# Autodesk Inventor assembly: Roof
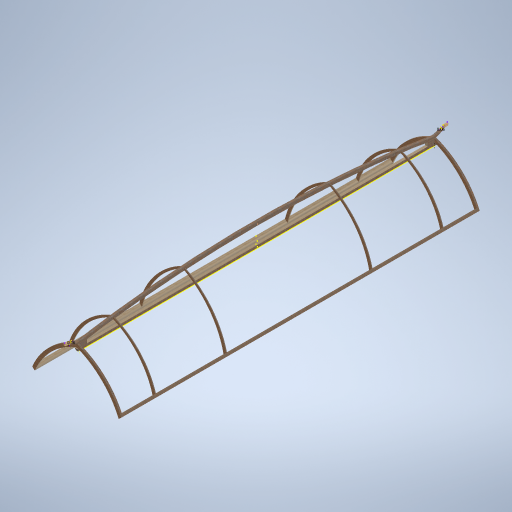
[picture p0: Inventor's stored thumbnail of the model, 512x512]
Saved by Autodesk Inventor 2024.2 (Build 282272000, 272)
## iProperties
Created: 2024-05-18
Part Number: Roof
Document SubType Name: Assembly
Designer: LOSTER_1
Author: LOSTER_1
## Documents named in this file (8)
- C:\Users\LOSTER_1\OneDrive\桌面\school\senior\Inventor_Project\ROOF\Roof.iam
- C:\Users\LOSTER_1\OneDrive\桌面\school\senior\Inventor_Project\ROOF\roof_beam.ipt
- C:\Users\LOSTER_1\OneDrive\桌面\school\senior\Inventor_Project\ROOF\gripping_beast.ipt
- C:\Users\LOSTER_1\OneDrive\桌面\school\senior\Inventor_Project\ROOF\main_crossbeam.ipt
- C:\Users\LOSTER_1\OneDrive\桌面\school\senior\Inventor_Project\ROOF\outer_curve_beam.ipt
- C:\Users\LOSTER_1\OneDrive\桌面\school\senior\Inventor_Project\ROOF\roof_straight_beam.ipt
- C:\Users\LOSTER_1\OneDrive\桌面\school\senior\Inventor_Project\ROOF\curve_beam_01.ipt
- C:\Users\LOSTER_1\OneDrive\桌面\school\senior\Inventor_Project\ROOF\curve_beam_02.ipt
## Components (18 placed, 7 different names)
1. roof_beam:1 — Mate:1, Mate:2, Mate:3, Mate:4, Mate:5, Mate:6, Mate:7, Mate:8, Mate:31, Mate:32, Mate:33, Mate:34, Mate:35, Mate:36, Mate:37, Mate:38, Mate:39, Mate:40, Mate:41, Mate:42, Mate:43, Mate:44, Mate:45, Mate:46, Mate:47, Mate:48, Mate:49, Mate:50
2. gripping_beast:1 — Mate:1, Mate:2, Mate:3, Mate:4
3. gripping_beast:2 — Mate:5
4. main_crossbeam:1 — Mate:6, Mate:7, Mate:8, Mate:11, Mate:14, Mate:19, Mate:20, Mate:21, Mate:22
5. outer_curve_beam:1 — Mate:9, Mate:10, Mate:11, Mate:12, Mate:13, Mate:26, Mate:28
6. outer_curve_beam:2 — Mate:9, Mate:10, Mate:12, Mate:13, Mate:14, Mate:29, Mate:30
7. outer_curve_beam:3 — Mate:23, Mate:24, Mate:25, Mate:27
8. outer_curve_beam:4 — Mate:19, Mate:20, Mate:21, Mate:22, Mate:23, Mate:24, Mate:25
9. roof_straight_beam:1 — Mate:26, Mate:27, Mate:28
10. roof_straight_beam:2 — Mate:29, Mate:30
11. curve_beam_01:1 — Mate:31, Mate:32, Mate:33
12. curve_beam_01:2 — Mate:34, Mate:35
13. curve_beam_01:3 — Mate:36, Mate:37
14. curve_beam_01:4 — Mate:38, Mate:39
15. curve_beam_02:1 — Mate:43, Mate:44
16. curve_beam_02:2 — Mate:40, Mate:41, Mate:42
17. curve_beam_02:3 — Mate:45, Mate:46, Mate:47
18. curve_beam_02:4 — Mate:48, Mate:49, Mate:50
## Relationships (50: Mate 50)
- Mate:1: roof_beam:1 ↔ gripping_beast:1
- Mate:2: roof_beam:1 ↔ gripping_beast:1
- Mate:3: roof_beam:1 ↔ gripping_beast:1
- Mate:4: roof_beam:1 ↔ gripping_beast:1
- Mate:5: roof_beam:1 ↔ gripping_beast:2
- Mate:6: roof_beam:1 ↔ main_crossbeam:1
- Mate:7: roof_beam:1 ↔ main_crossbeam:1
- Mate:8: roof_beam:1 ↔ main_crossbeam:1
- Mate:9: outer_curve_beam:1 ↔ outer_curve_beam:2
- Mate:10: outer_curve_beam:1 ↔ outer_curve_beam:2
- Mate:11: main_crossbeam:1 ↔ outer_curve_beam:1
- Mate:12: outer_curve_beam:1 ↔ outer_curve_beam:2
- Mate:13: outer_curve_beam:1 ↔ outer_curve_beam:2
- Mate:14: main_crossbeam:1 ↔ outer_curve_beam:2
- [Mate]: outer_curve_beam:3 ↔ outer_curve_beam:4
- [Mate]: outer_curve_beam:3 ↔ outer_curve_beam:4
- [Mate]: outer_curve_beam:3 ↔ outer_curve_beam:4
- [Mate]: outer_curve_beam:3 ↔ outer_curve_beam:4
- Mate:19: main_crossbeam:1 ↔ outer_curve_beam:4
- Mate:20: main_crossbeam:1 ↔ outer_curve_beam:4
- Mate:21: main_crossbeam:1 ↔ outer_curve_beam:4
- Mate:22: main_crossbeam:1 ↔ outer_curve_beam:4
- Mate:23: outer_curve_beam:3 ↔ outer_curve_beam:4
- Mate:24: outer_curve_beam:3 ↔ outer_curve_beam:4
- Mate:25: outer_curve_beam:3 ↔ outer_curve_beam:4
- Mate:26: outer_curve_beam:1 ↔ roof_straight_beam:1
- Mate:27: outer_curve_beam:3 ↔ roof_straight_beam:1
- Mate:28: outer_curve_beam:1 ↔ roof_straight_beam:1
- Mate:29: outer_curve_beam:2 ↔ roof_straight_beam:2
- Mate:30: outer_curve_beam:2 ↔ roof_straight_beam:2
- Mate:31: roof_beam:1 ↔ curve_beam_01:1
- Mate:32: roof_beam:1 ↔ curve_beam_01:1
- Mate:33: roof_beam:1 ↔ curve_beam_01:1
- Mate:34: roof_beam:1 ↔ curve_beam_01:2
- Mate:35: roof_beam:1 ↔ curve_beam_01:2
- Mate:36: roof_beam:1 ↔ curve_beam_01:3
- Mate:37: roof_beam:1 ↔ curve_beam_01:3
- Mate:38: roof_beam:1 ↔ curve_beam_01:4
- Mate:39: roof_beam:1 ↔ curve_beam_01:4
- Mate:40: roof_beam:1 ↔ curve_beam_02:2
- Mate:41: roof_beam:1 ↔ curve_beam_02:2
- Mate:42: roof_beam:1 ↔ curve_beam_02:2
- Mate:43: roof_beam:1 ↔ curve_beam_02:1
- Mate:44: roof_beam:1 ↔ curve_beam_02:1
- Mate:45: roof_beam:1 ↔ curve_beam_02:3
- Mate:46: roof_beam:1 ↔ curve_beam_02:3
- Mate:47: roof_beam:1 ↔ curve_beam_02:3
- Mate:48: roof_beam:1 ↔ curve_beam_02:4
- Mate:49: roof_beam:1 ↔ curve_beam_02:4
- Mate:50: roof_beam:1 ↔ curve_beam_02:4
## Named parameters: d16_d10 = 0 mm, d17_d11 = 0 mm, d18_d13 = 0 mm, d19_d14 = 0 mm
